# Autodesk Inventor assembly: Robot-ver4-1111-2020
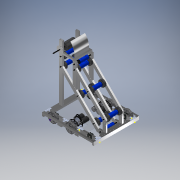
[picture p0: Inventor's stored thumbnail of the model, 180x180]
Saved by Autodesk Inventor 2018 (Build 220112000, 112)
## iProperties
Created: 2019-10-10
Part Number: Robot-ver4-1111-2020
Document SubType Name: Assembly
Designer: JMHal
Author: JMHal
## Documents named in this file (8)
- E:\GrabCAD\Power Hawks CAD\2020 Infinite Recharge\Final Robot Assembly\Robot-ver4-1111-2020.iam
- E:\GrabCAD\Power Hawks CAD\2020 Infinite Recharge\Chassis\Parts\Bumbers.ver1-1111-2019.ipt
- E:\GrabCAD\Power Hawks CAD\2020 Infinite Recharge\Chassis\Parts\BumperMount1-ver1-1111-2019.ipt
- E:\GrabCAD\Power Hawks CAD\2020 Infinite Recharge\Platform.ver1-1111-2020.ipt
- E:\GrabCAD\Power Hawks CAD\2020 Infinite Recharge\Powercell.ver1-1111-2020.ipt
- E:\GrabCAD\Power Hawks CAD\2020 Infinite Recharge\Lift\Assemblies\PistonLift-ver1-1111-2020.iam
- E:\GrabCAD\Power Hawks CAD\2020 Infinite Recharge\Final Robot Assembly\Shooter-Storage-IntakeAssembly.ver-1111-2020.iam
- E:\GrabCAD\Power Hawks CAD\2020 Infinite Recharge\Chassis\Assembly\Chassis-ver15-1111-2020.iam
## Components (8 placed, 7 different names)
1. Platform.ver1-1111-2020:1 — Tangent:2
2. Powercell.ver1-1111-2020:1 — Tangent:2
3. PistonLift-ver1-1111-2020:1 [sub-assembly] — Angle:24
4. Shooter-Storage-IntakeAssembly.ver-1111-2020:1 [sub-assembly]
5. Chassis-ver15-1111-2020:1 [sub-assembly]
6. Bumbers.ver1-1111-2019:1 — Mate:210
7. BumperMount1-ver1-1111-2019:2 — Mate:210
8. BumperMount1-ver1-1111-2019:3 — Angle:24
## Relationships (17: Mate 11, Flush 3, Tangent 2, Angle 1)
- [Mate] (-127 mm): Chassis-ver15-1111-2020:1 ↔ Bumbers.ver1-1111-2019:1
- [Mate]: Chassis-ver15-1111-2020:1 ↔ Bumbers.ver1-1111-2019:1
- [Mate]: Chassis-ver15-1111-2020:1 ↔ BumperMount1-ver1-1111-2019:2
- [Mate]: Chassis-ver15-1111-2020:1 ↔ BumperMount1-ver1-1111-2019:2
- [Mate]: Chassis-ver15-1111-2020:1 ↔ BumperMount1-ver1-1111-2019:2
- [Mate]: Chassis-ver15-1111-2020:1 ↔ BumperMount1-ver1-1111-2019:3
- [Mate]: Chassis-ver15-1111-2020:1 ↔ BumperMount1-ver1-1111-2019:3
- Mate:210: Bumbers.ver1-1111-2019:1 ↔ BumperMount1-ver1-1111-2019:2
- [Tangent]: Platform.ver1-1111-2020:1 ↔ Chassis-ver15-1111-2020:1
- Tangent:2: Platform.ver1-1111-2020:1 ↔ Powercell.ver1-1111-2020:1
- [Mate]: PistonLift-ver1-1111-2020:1 ↔ Chassis-ver15-1111-2020:1
- Angle:24 (0 deg): PistonLift-ver1-1111-2020:1 ↔ BumperMount1-ver1-1111-2019:3
- [Flush]: PistonLift-ver1-1111-2020:1 ↔ Chassis-ver15-1111-2020:1
- [Mate]: Shooter-Storage-IntakeAssembly.ver-1111-2020:1 ↔ Chassis-ver15-1111-2020:1
- [Mate]: Shooter-Storage-IntakeAssembly.ver-1111-2020:1 ↔ Chassis-ver15-1111-2020:1
- [Flush]: Shooter-Storage-IntakeAssembly.ver-1111-2020:1 ↔ Chassis-ver15-1111-2020:1
- [Flush]: PistonLift-ver1-1111-2020:1 ↔ Chassis-ver15-1111-2020:1
